# Autodesk Inventor assembly: OdroidAssembly
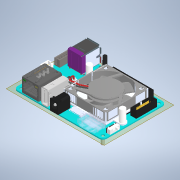
[picture p0: Inventor's stored thumbnail of the model, 180x180]
Saved by Autodesk Inventor 2020 (Build 240168000, 168)
## iProperties
Created: 2019-06-15
Part Number: OdroidAssembly
Document SubType Name: Assembly
Designer: amirt
Author: amirt
## Documents named in this file (3)
- C:\Users\amirt\Documents\Inventor\Drone\3DPrint\OdroidAssembly.iam
- C:\Users\amirt\Documents\Inventor\Drone\Imported Components\Odroid-XU4 v1.ipt
- C:\Users\amirt\Documents\Inventor\Drone\3DPrint\odroidstandoff.ipt
## Components (2 placed, 2 different names)
1. Odroid-XU4 v1:1 — Flush:1, Flush:2
2. odroidstandoff:1 — Flush:1, Flush:2
## Relationships (2: Flush 2)
- Flush:1: Odroid-XU4 v1:1 ↔ odroidstandoff:1
- Flush:2: Odroid-XU4 v1:1 ↔ odroidstandoff:1
